# Autodesk Inventor assembly: MainAssembly
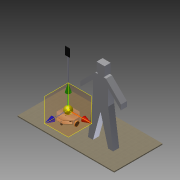
[picture p0: Inventor's stored thumbnail of the model, 180x180]
Saved by Autodesk Inventor 2012 (Build 160160000, 160)
## iProperties
Created: 2013-07-14
Part Number: MainAssembly
Document SubType Name: Assembly
Designer: joe_000
Mass: 5915.25 g
Surface Area: 98909.9 cm^2
Volume: 183567 cm^3
Density: 0.0322239 g/cm^3
Author: joe_000
## Documents named in this file (15)
- C:\dev\telepresenceRobot\mechanical\MainAssembly.iam
- C:\dev\telepresenceRobot\mechanical\Robot-Lower-Base.ipt
- C:\dev\telepresenceRobot\mechanical\MotorWheelAssembly.iam
- C:\dev\telepresenceRobot\mechanical\TB1230-Battery.ipt
- C:\dev\telepresenceRobot\mechanical\Robot-Upper-Base.ipt
- C:\dev\telepresenceRobot\mechanical\Robot-Mast.ipt
- C:\dev\telepresenceRobot\mechanical\Robot-Base-Support.ipt
- C:\dev\telepresenceRobot\mechanical\Robot-Base-BatteryBack.ipt
- C:\dev\telepresenceRobot\mechanical\Robot-Battery-Rails.ipt
- C:\dev\telepresenceRobot\mechanical\Human_5ft_9in.ipt
- C:\dev\telepresenceRobot\mechanical\Nexus7.ipt
- C:\dev\telepresenceRobot\mechanical\Robot-Base-Mast-Support.ipt
- C:\dev\telepresenceRobot\mechanical\Ground.ipt
- C:\dev\telepresenceRobot\mechanical\90973A120-Stainless Steel Tee Nut.ipt
- C:\dev\telepresenceRobot\mechanical\2834T190-Threaded-Stem Swivel Caster.ipt
## Components (22 placed, 14 different names)
1. Robot-Lower-Base:1 — Mate:1, Mate:2, Insert:1, Insert:2, Insert:3, Insert:4, Flush:1, Flush:2, Mate:6, Mate:7, Mate:8, Mate:15, Mate:16, Flush:3, Flush:4, Mate:19, Mate:20, Mate:22, Mate:29, Mate:30, Mate:31, Mate:32, Mate:38, Mate:39, Mate:44, Mate:49, Flush:9, Insert:7, Insert:8
2. MotorWheelAssembly:1 [sub-assembly] — Mate:2, Insert:2, Insert:3, Tangent:1
3. MotorWheelAssembly:2 [sub-assembly] — Mate:1, Insert:1, Insert:4
4. TB1230-Battery:1 — Mate:39, Mate:41, Mate:42
5. TB1230-Battery:2 — Mate:38, Mate:40, Mate:43
6. Robot-Upper-Base:1 — Flush:1, Flush:2, Mate:21
7. Robot-Mast:1 — Mate:6, Mate:7, Mate:8, Flush:8, Mate:47, Mate:48, Mate:50, Mate:51, Mate:53
8. Robot-Base-Support:1 — Mate:16, Flush:4, Mate:20, Mate:21, Mate:45, Flush:6
9. Robot-Base-Support:3 — Mate:15, Flush:3, Mate:19, Mate:23
10. Robot-Base-BatteryBack:1 — Mate:22, Mate:23, Mate:25, Mate:26, Mate:27, Mate:28, Mate:40, Mate:41, Mate:44
11. Robot-Battery-Rails:1 — Mate:28, Mate:31, Mate:35, Mate:43, Mate:47
12. Robot-Battery-Rails:2 — Mate:27, Mate:29, Mate:37, Mate:42, Mate:48
13. Robot-Battery-Rails:3 — Mate:26, Mate:30, Mate:37
14. Robot-Battery-Rails:4 — Mate:25, Mate:32, Mate:35
15. Human_5ft_9in:1 — Mate:45, Flush:6, Mate:52
16. Nexus7:1 — Flush:8, Mate:53
17. Robot-Base-Mast-Support:1 — Mate:49, Mate:50, Mate:51
18. Ground:1 — Tangent:1, Mate:52, Flush:9
19. 90973A120-Stainless Steel Tee Nut:1 — Insert:5, Insert:7
20. 90973A120-Stainless Steel Tee Nut:2 — Insert:6, Insert:8
21. 2834T190-Threaded-Stem Swivel Caster:1 — Insert:5
22. 2834T190-Threaded-Stem Swivel Caster:2 — Insert:6
## Relationships (53: Mate 37, Insert 8, Flush 7, Tangent 1)
- Mate:1: Robot-Lower-Base:1 ↔ MotorWheelAssembly:2
- Mate:2: Robot-Lower-Base:1 ↔ MotorWheelAssembly:1
- Insert:1: Robot-Lower-Base:1 ↔ MotorWheelAssembly:2
- Insert:2: Robot-Lower-Base:1 ↔ MotorWheelAssembly:1
- Insert:3: Robot-Lower-Base:1 ↔ MotorWheelAssembly:1
- Insert:4: Robot-Lower-Base:1 ↔ MotorWheelAssembly:2
- Flush:1: Robot-Lower-Base:1 ↔ Robot-Upper-Base:1
- Flush:2: Robot-Lower-Base:1 ↔ Robot-Upper-Base:1
- Mate:6: Robot-Lower-Base:1 ↔ Robot-Mast:1
- Mate:7: Robot-Lower-Base:1 ↔ Robot-Mast:1
- Mate:8: Robot-Lower-Base:1 ↔ Robot-Mast:1
- Mate:15: Robot-Lower-Base:1 ↔ Robot-Base-Support:3
- Mate:16: Robot-Lower-Base:1 ↔ Robot-Base-Support:1
- Flush:3: Robot-Lower-Base:1 ↔ Robot-Base-Support:3
- Flush:4: Robot-Lower-Base:1 ↔ Robot-Base-Support:1
- Mate:19: Robot-Lower-Base:1 ↔ Robot-Base-Support:3
- Mate:20: Robot-Lower-Base:1 ↔ Robot-Base-Support:1
- Mate:21: Robot-Upper-Base:1 ↔ Robot-Base-Support:1
- Mate:22: Robot-Lower-Base:1 ↔ Robot-Base-BatteryBack:1
- Mate:23: Robot-Base-Support:3 ↔ Robot-Base-BatteryBack:1
- Mate:25: Robot-Base-BatteryBack:1 ↔ Robot-Battery-Rails:4
- Mate:26: Robot-Base-BatteryBack:1 ↔ Robot-Battery-Rails:3
- Mate:27: Robot-Base-BatteryBack:1 ↔ Robot-Battery-Rails:2
- Mate:28: Robot-Base-BatteryBack:1 ↔ Robot-Battery-Rails:1
- Mate:29: Robot-Lower-Base:1 ↔ Robot-Battery-Rails:2
- Mate:30: Robot-Lower-Base:1 ↔ Robot-Battery-Rails:3
- Mate:31: Robot-Lower-Base:1 ↔ Robot-Battery-Rails:1
- Mate:32: Robot-Lower-Base:1 ↔ Robot-Battery-Rails:4
- Mate:35 (61.5875 mm): Robot-Battery-Rails:1 ↔ Robot-Battery-Rails:4
- Mate:37 (61.5875 mm): Robot-Battery-Rails:2 ↔ Robot-Battery-Rails:3
- Mate:38: Robot-Lower-Base:1 ↔ TB1230-Battery:2
- Mate:39: Robot-Lower-Base:1 ↔ TB1230-Battery:1
- Mate:40: TB1230-Battery:2 ↔ Robot-Base-BatteryBack:1
- Mate:41: TB1230-Battery:1 ↔ Robot-Base-BatteryBack:1
- Mate:42: TB1230-Battery:1 ↔ Robot-Battery-Rails:2
- Mate:43: TB1230-Battery:2 ↔ Robot-Battery-Rails:1
- Mate:44 (67 mm): Robot-Lower-Base:1 ↔ Robot-Base-BatteryBack:1
- Mate:45 (508 mm): Robot-Base-Support:1 ↔ Human_5ft_9in:1
- Flush:6: Robot-Base-Support:1 ↔ Human_5ft_9in:1
- Flush:8 (-50.8 mm): Robot-Mast:1 ↔ Nexus7:1
- Mate:47 (50.8 mm): Robot-Mast:1 ↔ Robot-Battery-Rails:1
- Mate:48 (50.8 mm): Robot-Mast:1 ↔ Robot-Battery-Rails:2
- Mate:49: Robot-Lower-Base:1 ↔ Robot-Base-Mast-Support:1
- Mate:50: Robot-Mast:1 ↔ Robot-Base-Mast-Support:1
- Mate:51: Robot-Mast:1 ↔ Robot-Base-Mast-Support:1
- Tangent:1: MotorWheelAssembly:1 ↔ Ground:1
- Mate:52: Human_5ft_9in:1 ↔ Ground:1
- Flush:9 (304.8 mm): Robot-Lower-Base:1 ↔ Ground:1
- Mate:53: Robot-Mast:1 ↔ Nexus7:1
- Insert:5 (4.572 mm): 90973A120-Stainless Steel Tee Nut:1 ↔ 2834T190-Threaded-Stem Swivel Caster:1
- Insert:6 (4.572 mm): 90973A120-Stainless Steel Tee Nut:2 ↔ 2834T190-Threaded-Stem Swivel Caster:2
- Insert:7: Robot-Lower-Base:1 ↔ 90973A120-Stainless Steel Tee Nut:1
- Insert:8: Robot-Lower-Base:1 ↔ 90973A120-Stainless Steel Tee Nut:2
## Named parameters: BatteryHeight = 60 mm, BatteryWidth = 66 mm, BatteryLength = 134 mm, CasterHeight = 4.572 mm
